# Autodesk Inventor assembly: 23-225
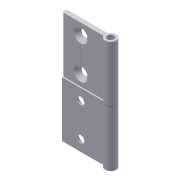
[picture p0: Inventor's stored thumbnail of the model, 180x180]
Saved by Autodesk Inventor 2011 SP2 (Build 150309200, 309)
## iProperties
Created: 2011-01-12
Part Number: 23-225
Document SubType Name: Assembly
Designer: dc85560
Stock Number: 23-225
Mass: 62.7007 g
Surface Area: 142.786 cm^2
Volume: 20.2347 cm^3
Density: 3.09867 g/cm^3
Title: Concealed Hinge 40
Author: dc85560
## Documents named in this file (3)
- R:\PSD 3 Library Update\IPS Part Files\05-Handles_Hinges\09-Conceled Hinge\23-225.iam
- R:\PSD 3 Library Update\IPS Part Files\05-Handles_Hinges\09-Conceled Hinge\23-225Z2.ipt
- R:\PSD 3 Library Update\IPS Part Files\05-Handles_Hinges\09-Conceled Hinge\23-225Z1.ipt
## Components (3 placed, 2 different names)
1. 23-225Z1:1 — Insert:1
2. 23-225Z2:1 — Insert:1, Insert:2
3. 23-225Z1:2 — Insert:2
## Relationships (2: Insert 2)
- Insert:1: 23-225Z1:1 ↔ 23-225Z2:1
- Insert:2: 23-225Z2:1 ↔ 23-225Z1:2
